# Autodesk Inventor assembly: TopChassis
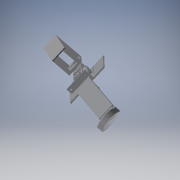
[picture p0: Inventor's stored thumbnail of the model, 180x180]
Saved by Autodesk Inventor 2016 (Build 200138000, 138)
## iProperties
Created: 2016-05-07
Part Number: TopChassis
Document SubType Name: Assembly
Designer: mkepler
Author: mkepler
## Documents named in this file (7)
- C:\Users\mkepler\Google Drive\Michael Kepler\College\ECE\ECE 590\Final Project\Mechanical Design\Inventor Files\TopChassis.iam
- C:\Users\mkepler\Google Drive\Michael Kepler\College\ECE\ECE 590\Final Project\Mechanical Design\Inventor Files\cameraMount.ipt
- C:\Users\mkepler\Google Drive\Michael Kepler\College\ECE\ECE 590\Final Project\Mechanical Design\Inventor Files\cup.ipt
- C:\Users\mkepler\Google Drive\Michael Kepler\College\ECE\ECE 590\Final Project\Mechanical Design\Inventor Files\leverArm.ipt
- C:\Users\mkepler\Google Drive\Michael Kepler\College\ECE\ECE 590\Final Project\Mechanical Design\Inventor Files\leverServoMount.ipt
- C:\Users\mkepler\Google Drive\Michael Kepler\College\ECE\ECE 590\Final Project\Mechanical Design\Inventor Files\topChassis.ipt
- C:\Users\mkepler\Google Drive\Michael Kepler\College\ECE\ECE 590\Final Project\Mechanical Design\Inventor Files\xl320Servo.ipt
## Components (7 placed, 6 different names)
1. cameraMount:1 — Insert:11, Insert:12
2. cup:1 — Insert:6, Insert:7
3. leverArm:1 — Insert:4, Insert:5, Insert:6, Insert:7
4. leverServoMount:1 — Insert:4, Insert:5, Insert:9, Insert:10
5. topChassis:1 — Insert:1, Insert:2, Insert:8
6. xl320Servo:1 — Insert:1, Insert:2, Insert:9, Insert:10
7. xl320Servo:2 — Insert:8, Insert:11, Insert:12
## Relationships (11: Insert 11)
- Insert:1: topChassis:1 ↔ xl320Servo:1
- Insert:2: topChassis:1 ↔ xl320Servo:1
- Insert:4: leverArm:1 ↔ leverServoMount:1
- Insert:5: leverArm:1 ↔ leverServoMount:1
- Insert:6: cup:1 ↔ leverArm:1
- Insert:7: cup:1 ↔ leverArm:1
- Insert:8: topChassis:1 ↔ xl320Servo:2
- Insert:9: leverServoMount:1 ↔ xl320Servo:1
- Insert:10: leverServoMount:1 ↔ xl320Servo:1
- Insert:11: cameraMount:1 ↔ xl320Servo:2
- Insert:12: cameraMount:1 ↔ xl320Servo:2
